# Autodesk Inventor assembly: 사각형 OV-PAM 10패턴
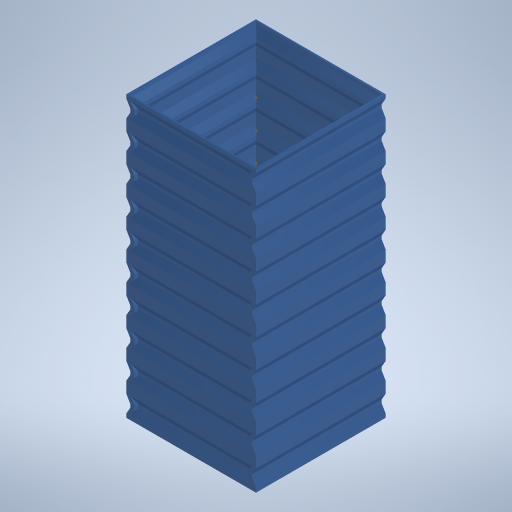
[picture p0: Inventor's stored thumbnail of the model, 512x512]
Saved by Autodesk Inventor 2024 (Build 280153000, 153)
## iProperties
Created: 2023-06-16
Part Number: 사각형 OV-PAM 10패턴
Document SubType Name: Assembly
Designer: jsw
Author: jsw
## Documents named in this file (3)
- C:\승원\co-op\OV-PAM\사각형 OV-PAM 10패턴.iam
- C:\승원\co-op\OV-PAM\사각형 OV-PAM 10패턴 층 중단 하단 연결 층.ipt
- C:\승원\co-op\OV-PAM\사각형 OV-PAM 10패턴 층 한개.ipt
## Components (10 placed, 2 different names)
1. 사각형 OV-PAM 10패턴 층 중단 하단 연결 층:1 — 메이트:1, 플러쉬:1, 플러쉬:2
2. 사각형 OV-PAM 10패턴 층 중단 하단 연결 층:2 — 메이트:2, 플러쉬:3, 플러쉬:4
3. 사각형 OV-PAM 10패턴 층 한개:1 — 메이트:1, 플러쉬:1, 플러쉬:2
4. 사각형 OV-PAM 10패턴 층 한개:2
5. 사각형 OV-PAM 10패턴 층 한개:3
6. 사각형 OV-PAM 10패턴 층 한개:4
7. 사각형 OV-PAM 10패턴 층 한개:5
8. 사각형 OV-PAM 10패턴 층 한개:6
9. 사각형 OV-PAM 10패턴 층 한개:7
10. 사각형 OV-PAM 10패턴 층 한개:8 — 메이트:2, 플러쉬:3, 플러쉬:4
## Component patterns: (8 elements, first: 사각형 OV-PAM 10패턴 층 한개:1)
## Relationships (6: Flush 4, Mate 2)
- 메이트:1 [Mate]: 사각형 OV-PAM 10패턴 층 중단 하단 연결 층:1 ↔ 사각형 OV-PAM 10패턴 층 한개:1
- 플러쉬:1 [Flush]: 사각형 OV-PAM 10패턴 층 중단 하단 연결 층:1 ↔ 사각형 OV-PAM 10패턴 층 한개:1
- 플러쉬:2 [Flush]: 사각형 OV-PAM 10패턴 층 중단 하단 연결 층:1 ↔ 사각형 OV-PAM 10패턴 층 한개:1
- 메이트:2 [Mate]: 사각형 OV-PAM 10패턴 층 중단 하단 연결 층:2 ↔ 사각형 OV-PAM 10패턴 층 한개:8
- 플러쉬:3 [Flush]: 사각형 OV-PAM 10패턴 층 중단 하단 연결 층:2 ↔ 사각형 OV-PAM 10패턴 층 한개:8
- 플러쉬:4 [Flush]: 사각형 OV-PAM 10패턴 층 중단 하단 연결 층:2 ↔ 사각형 OV-PAM 10패턴 층 한개:8
